# Autodesk Inventor assembly: Shooter Motor
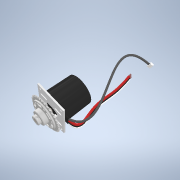
[picture p0: Inventor's stored thumbnail of the model, 180x180]
Saved by Autodesk Inventor 2020 (Build 240168000, 168)
## iProperties
Created: 2020-02-03
Part Number: Shooter Motor
Document SubType Name: Assembly
Designer: JimAndVal
Author: JimAndVal
## Documents named in this file (4)
- D:\Users\JimAndVal\Documents\JIM\IronRiders\2020 Robot-1\Manipulators\Hooded Shooter (Protected Zone)\Shooter Motor.iam
- D:\Users\JimAndVal\Documents\JIM\IronRiders\2020 Robot-1\Manipulators\Hooded Shooter (Protected Zone)\NEO.ipt
- D:\Users\JimAndVal\Documents\JIM\IronRiders\2020 Robot-1\Manipulators\Hooded Shooter (Protected Zone)\34 tooth gear for 8 mm shaft.iam
- D:\Users\JimAndVal\Documents\JIM\IronRiders\2020 Robot-1\Manipulators\Hooded Shooter (Protected Zone)\Neo Mounting Plate.ipt
## Components (3 placed, 3 different names)
1. NEO:1 — Mate:3, Mate:4, Mate:5, Flush:4
2. 34 tooth gear for 8 mm shaft:1 [sub-assembly] — Mate:5, Flush:4
3. Neo Mounting Plate:1 — Flush:2
## Relationships (7: Mate 4, Flush 3)
- [Mate]: NEO:1 ↔ Neo Mounting Plate:1
- Flush:2 (-38.1 mm): Neo Mounting Plate:1
- Flush:3 (17.9578 mm)
- Mate:3: NEO:1
- Mate:4: NEO:1
- Mate:5: NEO:1 ↔ 34 tooth gear for 8 mm shaft:1
- Flush:4: NEO:1 ↔ 34 tooth gear for 8 mm shaft:1
